# Autodesk Inventor assembly: Full Robot
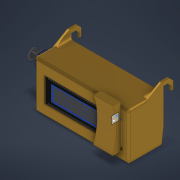
[picture p0: Inventor's stored thumbnail of the model, 180x180]
Saved by Autodesk Inventor 2022 (Build 260153000, 153)
## iProperties
Created: 2021-08-06
Part Number: Full Robot
Document SubType Name: Assembly
Designer: sidsa
Author: sidsa
## Documents named in this file (5)
- D:\My Documents\gitHUB Rocketry\mlh-robo-hacks\Inventor CAD\Full Robot.iam
- D:\My Documents\gitHUB Rocketry\mlh-robo-hacks\Inventor CAD\Electronics\20x4 LCD\ERM2004-2_3D.ipt
- D:\My Documents\gitHUB Rocketry\mlh-robo-hacks\Inventor CAD\Electronics\Joystick\Joystick HW504 Board.ipt
- D:\My Documents\gitHUB Rocketry\mlh-robo-hacks\Inventor CAD\Mount Case.ipt
- D:\My Documents\gitHUB Rocketry\mlh-robo-hacks\Inventor CAD\LED Reflector.ipt
## Components (4 placed, 4 different names)
1. ERM2004-2_3D:1 — Mate:2
2. Joystick HW504 Board:1 — Mate:3
3. Mount Case:1 — Mate:2, Mate:3, Mate:4
4. LED Reflector:1 — Mate:4
## Relationships (3: Mate 3)
- Mate:2: ERM2004-2_3D:1 ↔ Mount Case:1
- Mate:3: Joystick HW504 Board:1 ↔ Mount Case:1
- Mate:4: Mount Case:1 ↔ LED Reflector:1
